# Autodesk Inventor assembly: BungaCamp
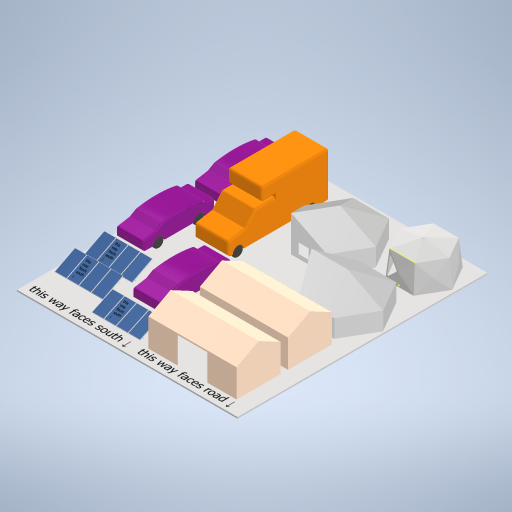
[picture p0: Inventor's stored thumbnail of the model, 512x512]
Saved by Autodesk Inventor 2023 (Build 270158000, 158)
## iProperties
Created: 2024-07-15
Part Number: BungaCamp
Document SubType Name: Assembly
Designer: incep
Author: incep
## Documents named in this file (8)
- C:\Projects\BungaCamp\BungaCamp.iam
- C:\Projects\BungaCamp\BungaCamp-Layout.ipt
- C:\Projects\BungaCamp\BungaCamp-H13-Hexayurt-QTY2.ipt
- C:\Projects\BungaCamp\BungaCamp-CostcoCarport-QTY2.ipt
- C:\Projects\BungaCamp\BungaCamp-Uhaul15ft-QTY1.ipt
- C:\Projects\BungaCamp\BungaCamp-Sedan-QTY3.ipt
- C:\Projects\BungaCamp\BungaCamp-SolarArray1kW-QTY2.ipt
- C:\Projects\BungaCamp\BungaCamp-ShiftPod.ipt
## Components (13 placed, 7 different names)
1. BungaCamp-Layout:1 — Flush:1, Flush:2, Flush:3, Mate:1, Mate:2, Mate:3, Mate:4, Mate:5, Mate:6, Mate:7, Flush:4, Tangent:1, Tangent:2, Tangent:3, Mate:9, Mate:10, Tangent:4, Mate:11, Mate:12
2. BungaCamp-H13-Hexayurt-QTY2:1 — Mate:4, Mate:13
3. BungaCamp-H13-Hexayurt-QTY2:2 — Mate:5, Mate:13
4. BungaCamp-CostcoCarport-QTY2:1 — Mate:6, Mate:8, Flush:4, Flush:5
5. BungaCamp-CostcoCarport-QTY2:2 — Mate:7, Mate:8, Flush:5
6. BungaCamp-Uhaul15ft-QTY1:1 — Tangent:1
7. BungaCamp-Sedan-QTY3:1 — Tangent:2
8. BungaCamp-Sedan-QTY3:2 — Tangent:3
9. BungaCamp-SolarArray1kW-QTY2:1 — Mate:9, Flush:6
10. BungaCamp-SolarArray1kW-QTY2:2 — Mate:10, Flush:6
11. BungaCamp-Sedan-QTY3:3 — Tangent:4
12. BungaCamp-SolarArray1kW-QTY2:3 — Mate:11
13. BungaCamp-ShiftPod:1 — Mate:12
## Relationships (23: Mate 13, Flush 6, Tangent 4)
- Flush:1: BungaCamp-Layout:1
- Flush:2: BungaCamp-Layout:1
- Flush:3: BungaCamp-Layout:1
- Mate:1: BungaCamp-Layout:1
- Mate:2: BungaCamp-Layout:1
- Mate:3: BungaCamp-Layout:1
- Mate:4: BungaCamp-Layout:1 ↔ BungaCamp-H13-Hexayurt-QTY2:1
- Mate:5: BungaCamp-Layout:1 ↔ BungaCamp-H13-Hexayurt-QTY2:2
- Mate:6: BungaCamp-Layout:1 ↔ BungaCamp-CostcoCarport-QTY2:1
- Mate:7: BungaCamp-Layout:1 ↔ BungaCamp-CostcoCarport-QTY2:2
- Mate:8 (500 mm): BungaCamp-CostcoCarport-QTY2:1 ↔ BungaCamp-CostcoCarport-QTY2:2
- Flush:4 (1000 mm): BungaCamp-Layout:1 ↔ BungaCamp-CostcoCarport-QTY2:1
- Flush:5: BungaCamp-CostcoCarport-QTY2:1 ↔ BungaCamp-CostcoCarport-QTY2:2
- Tangent:1: BungaCamp-Layout:1 ↔ BungaCamp-Uhaul15ft-QTY1:1
- Tangent:2: BungaCamp-Layout:1 ↔ BungaCamp-Sedan-QTY3:1
- Tangent:3: BungaCamp-Layout:1 ↔ BungaCamp-Sedan-QTY3:2
- Mate:9: BungaCamp-Layout:1 ↔ BungaCamp-SolarArray1kW-QTY2:1
- Mate:10: BungaCamp-Layout:1 ↔ BungaCamp-SolarArray1kW-QTY2:2
- Flush:6: BungaCamp-SolarArray1kW-QTY2:1 ↔ BungaCamp-SolarArray1kW-QTY2:2
- Tangent:4: BungaCamp-Layout:1 ↔ BungaCamp-Sedan-QTY3:3
- Mate:11: BungaCamp-Layout:1 ↔ BungaCamp-SolarArray1kW-QTY2:3
- Mate:12: BungaCamp-Layout:1 ↔ BungaCamp-ShiftPod:1
- Mate:13 (1000 mm): BungaCamp-H13-Hexayurt-QTY2:1 ↔ BungaCamp-H13-Hexayurt-QTY2:2
